# Autodesk Inventor assembly: Whole-Assembly
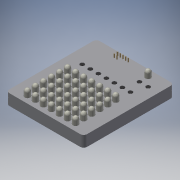
[picture p0: Inventor's stored thumbnail of the model, 180x180]
Saved by Autodesk Inventor 2018.3 (Build 223284000, 284)
## iProperties
Created: 2019-10-06
Part Number: Whole-Assembly
Document SubType Name: Assembly
Designer: Jamal Bouajjaj
Author: Jamal Bouajjaj
## Documents named in this file (4)
- F:\Projects\Connect4 Board\CAD\Whole-Assembly.iam
- F:\Projects\Connect4 Board\CAD\PCB-Assembly.iam
- F:\Projects\Connect4 Board\CAD\Buttom Part.ipt
- F:\Projects\Connect4 Board\CAD\Top Part.ipt
## Components (3 placed, 3 different names)
1. PCB-Assembly:1 [sub-assembly] — Mate:1, Mate:2, Mate:3, Mate:4, Mate:5, Mate:6
2. Buttom Part:1 — Mate:1, Mate:2, Mate:3
3. Top Part:1 — Mate:4, Mate:5, Mate:6
## Relationships (6: Mate 6)
- Mate:1: PCB-Assembly:1 ↔ Buttom Part:1
- Mate:2: PCB-Assembly:1 ↔ Buttom Part:1
- Mate:3: PCB-Assembly:1 ↔ Buttom Part:1
- Mate:4: PCB-Assembly:1 ↔ Top Part:1
- Mate:5: PCB-Assembly:1 ↔ Top Part:1
- Mate:6: PCB-Assembly:1 ↔ Top Part:1
